# Autodesk Inventor assembly: EFFECTOR
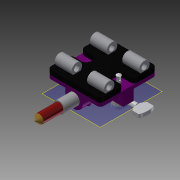
[picture p0: Inventor's stored thumbnail of the model, 180x180]
Saved by Autodesk Inventor 2013 (Build 170138000, 138)
## iProperties
Created: 2014-03-03
Part Number: EFFECTOR
Document SubType Name: Assembly
Designer: employee
Author: employee
## Documents named in this file (7)
- C:\Users\employee\Desktop\CoreXZ\EFFECTOR.iam
- C:\Users\employee\Desktop\CoreXZ\EFFECTOR BEARING PLATE.ipt
- C:\Users\employee\Desktop\CoreXZ\LM8UU.ipt
- C:\Users\employee\Desktop\CoreXZ\EFFECTOR SECONDARY PLATE.ipt
- C:\Users\employee\Desktop\CoreXZ\UBIS.ipt
- C:\Users\employee\Desktop\CoreXZ\TUNING PEG.ipt
- C:\Users\employee\Desktop\CoreXZ\M3X20.ipt
## Components (12 placed, 6 different names)
1. EFFECTOR BEARING PLATE:1 — Insert:1, Insert:2, Insert:3, Insert:4, Flush:1
2. LM8UU:1 — Insert:1
3. LM8UU:2 — Insert:2
4. LM8UU:3 — Insert:3
5. LM8UU:4 — Insert:4
6. EFFECTOR SECONDARY PLATE:1 — Flush:1, Insert:5, Angle:1, Mate:1, Mate:2, Insert:6, Insert:7, Insert:8, Insert:9
7. UBIS:1 — Insert:5
8. TUNING PEG:1 — Angle:1, Mate:1, Mate:2
9. M3X20:1 — Insert:8
10. M3X20:2 — Insert:6
11. M3X20:3 — Insert:7
12. M3X20:4 — Insert:9
## Relationships (13: Insert 9, Mate 2, Flush 1, Angle 1)
- Insert:1: EFFECTOR BEARING PLATE:1 ↔ LM8UU:1
- Insert:2: EFFECTOR BEARING PLATE:1 ↔ LM8UU:2
- Insert:3: EFFECTOR BEARING PLATE:1 ↔ LM8UU:3
- Insert:4: EFFECTOR BEARING PLATE:1 ↔ LM8UU:4
- Flush:1: EFFECTOR BEARING PLATE:1 ↔ EFFECTOR SECONDARY PLATE:1
- Insert:5: EFFECTOR SECONDARY PLATE:1 ↔ UBIS:1
- Angle:1 (0 deg): EFFECTOR SECONDARY PLATE:1 ↔ TUNING PEG:1
- Mate:1: EFFECTOR SECONDARY PLATE:1 ↔ TUNING PEG:1
- Mate:2: EFFECTOR SECONDARY PLATE:1 ↔ TUNING PEG:1
- Insert:6: EFFECTOR SECONDARY PLATE:1 ↔ M3X20:2
- Insert:7: EFFECTOR SECONDARY PLATE:1 ↔ M3X20:3
- Insert:8 (5 mm): EFFECTOR SECONDARY PLATE:1 ↔ M3X20:1
- Insert:9 (5 mm): EFFECTOR SECONDARY PLATE:1 ↔ M3X20:4
